# Autodesk Inventor assembly: Hoja Oculta
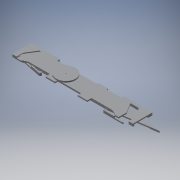
[picture p0: Inventor's stored thumbnail of the model, 180x180]
Saved by Autodesk Inventor 2016 (Build 200138000, 138)
## iProperties
Created: 2015-03-12
Part Number: Hoja Oculta
Document SubType Name: Assembly
Designer: amatiasq
Author: amatiasq
## Documents named in this file (12)
- C:\Users\amatiasq\Documents\GitHub\3D\Hoja Oculta\Optimizada\Hoja Oculta.iam
- C:\Users\amatiasq\Documents\GitHub\3D\Hoja Oculta\Optimizada\Base.ipt
- C:\Users\amatiasq\Documents\GitHub\3D\Hoja Oculta\Optimizada\Hoja.ipt
- C:\Users\amatiasq\Documents\GitHub\3D\Hoja Oculta\Optimizada\Deslizador.ipt
- C:\Users\amatiasq\Documents\GitHub\3D\Hoja Oculta\Optimizada\Traba.ipt
- C:\Users\amatiasq\Documents\GitHub\3D\Hoja Oculta\Optimizada\Traba_MIR.ipt
- C:\Users\amatiasq\Documents\GitHub\3D\Hoja Oculta\Optimizada\Tirador.ipt
- C:\Users\amatiasq\Documents\GitHub\3D\Hoja Oculta\Optimizada\Tirador_MIR.ipt
- C:\Users\amatiasq\Documents\GitHub\3D\Hoja Oculta\Optimizada\Rueda interna.ipt
- C:\Users\amatiasq\Documents\GitHub\3D\Hoja Oculta\Optimizada\Rueda externa.ipt
- C:\Users\amatiasq\Documents\GitHub\3D\Hoja Oculta\Optimizada\Tapa.ipt
- C:\Users\amatiasq\Documents\GitHub\3D\Hoja Oculta\Optimizada\Rueda superior.ipt
## Components (11 placed, 11 different names)
1. Base:1 — Hoja - Altura, Hoja - Movimiento, Hoja - Lateral, Deslizador - Altura, Deslizador - Lateral, Deslizador - Movimiento, Insertar:2, Insertar:3, Ángulo:1, Ángulo:2, Tirador trasero - Movimiento, Tirador trasero - Lateral, Tirador trasero - Base, Tirador delantero - Movimiento, Tirador delantero - Lateral, Tirador delantero - Base, Tapa - Altura, Tapa - Lateral, Tapa - Longitud
2. Hoja:1 — Hoja - Altura, Hoja - Movimiento, Hoja - Lateral, Tirador trasero - Hoja, Tirador delantero - Hoja
3. Deslizador:1 — Deslizador - Altura, Deslizador - Lateral, Deslizador - Movimiento, Tangente:1, Tangente:2, Tirador trasero - Deslizador, Tirador delantero - Deslizador, Rueda interna - Movimiento
4. Traba:1 — Insertar:3, Ángulo:1, Tangente:1
5. Traba_MIR:1 — Insertar:2, Ángulo:2, Tangente:2
6. Tirador:1 — Tirador trasero - Movimiento, Tirador trasero - Lateral, Tirador trasero - Hoja, Tirador trasero - Base, Tirador trasero - Deslizador
7. Tirador_MIR:1 — Tirador delantero - Movimiento, Tirador delantero - Lateral, Tirador delantero - Hoja, Tirador delantero - Base, Tirador delantero - Deslizador
8. Rueda interna:1 — Rueda interna - Movimiento, Rueda externa - interna - posicion, Rueda externa - interna - soldadura
9. Rueda externa:1 — Rueda externa - interna - posicion, Rueda externa - interna - soldadura, Rueda superior - externa, Rueda superior - externa - soldadura, Rueda externa - Tapa
10. Rueda superior:1 — Rueda superior - externa, Rueda superior - externa - soldadura
11. Tapa:1 — Tapa - Altura, Tapa - Lateral, Tapa - Longitud, Rueda externa - Tapa
## Relationships (31: Mate 19, Insert 5, Tangent 3, Angle 2, RelateRotation 2)
- Hoja - Altura [Mate] (0.3 mm): Base:1 ↔ Hoja:1
- Hoja - Movimiento [Mate]: Base:1 ↔ Hoja:1
- Hoja - Lateral [Mate] (0.3 mm): Base:1 ↔ Hoja:1
- Deslizador - Altura [Mate] (2.3 mm): Base:1 ↔ Deslizador:1
- Deslizador - Lateral [Mate] (0.3 mm): Base:1 ↔ Deslizador:1
- Deslizador - Movimiento [Mate]: Base:1 ↔ Deslizador:1
- Insertar:2: Base:1 ↔ Traba_MIR:1
- Insertar:3: Base:1 ↔ Traba:1
- Ángulo:1 [Angle] (163 deg): Base:1 ↔ Traba:1
- Tangente:1: Deslizador:1 ↔ Traba:1
- Ángulo:2 [Angle] (180 deg): Base:1 ↔ Traba_MIR:1
- Tangente:2: Deslizador:1 ↔ Traba_MIR:1
- Tirador trasero - Movimiento [Mate] (17 mm): Base:1 ↔ Tirador:1
- Tirador trasero - Lateral [Mate] (0.3 mm): Base:1 ↔ Tirador:1
- Tirador trasero - Hoja [Mate]: Hoja:1 ↔ Tirador:1
- Tirador trasero - Base [Mate]: Base:1 ↔ Tirador:1
- Tirador trasero - Deslizador [Mate]: Deslizador:1 ↔ Tirador:1
- Tirador delantero - Movimiento [Mate]: Base:1 ↔ Tirador_MIR:1
- Tirador delantero - Lateral [Mate] (0.3 mm): Base:1 ↔ Tirador_MIR:1
- Tirador delantero - Hoja [Mate]: Hoja:1 ↔ Tirador_MIR:1
- Tirador delantero - Base [Mate]: Base:1 ↔ Tirador_MIR:1
- Tirador delantero - Deslizador [Mate]: Deslizador:1 ↔ Tirador_MIR:1
- Rueda interna - Movimiento [Tangent] (0.15 mm): Deslizador:1 ↔ Rueda interna:1
- Rueda externa - interna - posicion [Insert]: Rueda interna:1 ↔ Rueda externa:1
- Tapa - Altura [Mate]: Base:1 ↔ Tapa:1
- Tapa - Lateral [Mate] (0.1 mm): Base:1 ↔ Tapa:1
- Tapa - Longitud [Mate] (0.1 mm): Base:1 ↔ Tapa:1
- Rueda externa - interna - soldadura [RelateRotation] (1.133 ul): Rueda interna:1 ↔ Rueda externa:1
- Rueda superior - externa [Insert]: Rueda externa:1 ↔ Rueda superior:1
- Rueda superior - externa - soldadura [RelateRotation] (1 ul): Rueda externa:1 ↔ Rueda superior:1
- Rueda externa - Tapa [Insert] (0.05 mm): Rueda externa:1 ↔ Tapa:1
